# Autodesk Inventor assembly: LeftShoulderBearingUnit
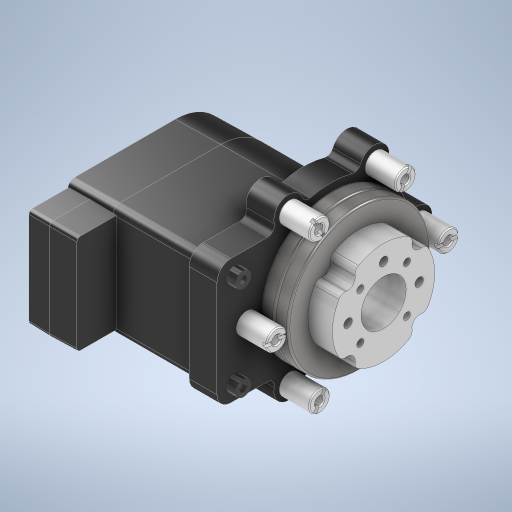
[picture p0: Inventor's stored thumbnail of the model, 512x512]
Saved by Autodesk Inventor 2024.2 (Build 282272000, 272)
## iProperties
Created: 2024-04-13
Part Number: LeftShoulderBearingUnit
Document SubType Name: Assembly
Designer: Masato Kubotera
Author: Masato Kubotera
## Documents named in this file (3)
- C:\Users\masato\OneDrive - Chiba Institute of Technology\CIT Brains\RoboCup2024\Mechanic\SUSTAINA-OP2-DEV - 作業\NativeFiles\Boby\UpperLimb\Shoulders\LeftShoulderBearingUnit.iam
- C:\Users\masato\OneDrive - Chiba Institute of Technology\CIT Brains\RoboCup2024\Mechanic\SUSTAINA-OP2-DEV - 作業\NativeFiles\Boby\UpperLimb\Shoulders\ShoulderBearingUnitBasis.iam
- C:\Users\masato\OneDrive - Chiba Institute of Technology\CIT Brains\RoboCup2024\Mechanic\SUSTAINA-OP2-DEV - 作業\NativeFiles\Boby\CommonDesignedComponents\CrossRollerBearingUnit\CrossRollerBearingInnerSupportStand.ipt
## Components (2 placed, 2 different names)
1. Shoulder_CrossRollerBearingUnit:1 [sub-assembly] — Flush:1, Flush:3, Flush:2, Insert:1
2. CrossRollerBearingInnerSupportStand:1 — Insert:1, Angle:1
## Relationships (5: Flush 3, Insert 1, Angle 1)
- Flush:1: Shoulder_CrossRollerBearingUnit:1
- Flush:3: Shoulder_CrossRollerBearingUnit:1
- Flush:2: Shoulder_CrossRollerBearingUnit:1
- Insert:1: Shoulder_CrossRollerBearingUnit:1 ↔ CrossRollerBearingInnerSupportStand:1
- Angle:1 (0 deg): CrossRollerBearingInnerSupportStand:1
